# Autodesk Inventor assembly: Hebel_Klemme
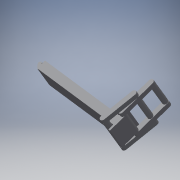
[picture p0: Inventor's stored thumbnail of the model, 180x180]
Saved by Autodesk Inventor 2018 (Build 220112000, 112)
## iProperties
Created: 2018-02-02
Part Number: Hebel_Klemme
Material: Generisch
Document SubType Name: Assembly
Designer: Julian
Author: Julian
## Documents named in this file (10)
- C:\Users\Julian\Desktop\Schule\5AHME\Diplomarbeit\Git\fuettr_prototype\Mechanical\Inventorskizzen\Hebel_Klemme.iam
- C:\Users\Julian\Desktop\Schule\5AHME\Diplomarbeit\Git\fuettr_prototype\Mechanical\Inventorskizzen\Hebel_KLemme_Hebel.ipt
- C:\Users\Julian\Desktop\Schule\5AHME\Diplomarbeit\Git\fuettr_prototype\Mechanical\Inventorskizzen\Hebel_Klemme_oben.ipt
- C:\Users\Julian\Desktop\Schule\5AHME\Diplomarbeit\Git\fuettr_prototype\Mechanical\Inventorskizzen\Hebel_Klemme_Rohrende.ipt
- C:\Users\Julian\Desktop\Schule\5AHME\Diplomarbeit\Git\fuettr_prototype\Mechanical\Inventorskizzen\Hebel_Klemme_unten.ipt
- C:\Users\Julian\Desktop\Schule\5AHME\Diplomarbeit\Git\fuettr_prototype\Mechanical\Inventorskizzen\Hebel_Röhre.ipt
- C:\Users\Julian\Desktop\Schule\5AHME\Diplomarbeit\Git\fuettr_prototype\Mechanical\Inventorskizzen\Klemme_Hebel_Entstück.ipt
- C:\Users\Julian\Desktop\Schule\5AHME\Diplomarbeit\Git\fuettr_prototype\Mechanical\Inventorskizzen\Stift_28mm.ipt
- C:\Users\Julian\Desktop\Schule\5AHME\Diplomarbeit\Git\fuettr_prototype\Mechanical\Inventorskizzen\Stift_20mm.ipt
- C:\Users\Julian\Desktop\Schule\5AHME\Diplomarbeit\Git\fuettr_prototype\Mechanical\Inventorskizzen\Stift_36mm.ipt
## Components (14 placed, 9 different names)
1. Hebel_KLemme_Hebel:1 — Drehbar:2, Starr:1, Drehbar:4, Drehbar:6, Drehbar:1, Starr:4, Starr:6
2. Hebel_KLemme_Hebel:2 — Drehbar:3, Drehbar:5
3. Hebel_Klemme_oben:1
4. Hebel_Klemme_Rohrende:1 — Starr:2, Starr:3
5. Hebel_Klemme_unten:1 — Drehbar:1, Drehbar:2, Drehbar:3, Starr:5
6. Hebel_Röhre:1 — Starr:1
7. Klemme_Hebel_Entstück:1 — Drehbar:5, Starr:2
8. Klemme_Hebel_Entstück:2 — Drehbar:4, Starr:3, Starr:7, Starr:8
9. Hebel_Röhre:2 — Drehbar:6
10. Stift_28mm:1 — Starr:4
11. Stift_20mm:1 — Starr:5
12. Stift_28mm:2 — Starr:6
13. Stift_36mm:1 — Starr:7
14. Stift_36mm:2 — Starr:8
## Relationships (14: WeldJoint 8, RevoluteJoint 6)
- Drehbar:1 [RevoluteJoint]: Hebel_KLemme_Hebel:1 ↔ Hebel_Klemme_unten:1
- Drehbar:2 [RevoluteJoint]: Hebel_KLemme_Hebel:1 ↔ Hebel_Klemme_unten:1
- Drehbar:3 [RevoluteJoint]: Hebel_KLemme_Hebel:2 ↔ Hebel_Klemme_unten:1
- Starr:1 [WeldJoint]: Hebel_KLemme_Hebel:1 ↔ Hebel_Röhre:1
- Drehbar:4 [RevoluteJoint]: Hebel_KLemme_Hebel:1 ↔ Klemme_Hebel_Entstück:2
- Drehbar:5 [RevoluteJoint]: Hebel_KLemme_Hebel:2 ↔ Klemme_Hebel_Entstück:1
- Starr:2 [WeldJoint]: Hebel_Klemme_Rohrende:1 ↔ Klemme_Hebel_Entstück:1
- Starr:3 [WeldJoint]: Hebel_Klemme_Rohrende:1 ↔ Klemme_Hebel_Entstück:2
- Drehbar:6 [RevoluteJoint]: Hebel_KLemme_Hebel:1 ↔ Hebel_Röhre:2
- Starr:4 [WeldJoint]: Hebel_KLemme_Hebel:1 ↔ Stift_28mm:1
- Starr:5 [WeldJoint]: Hebel_Klemme_unten:1 ↔ Stift_20mm:1
- Starr:6 [WeldJoint]: Hebel_KLemme_Hebel:1 ↔ Stift_28mm:2
- Starr:7 [WeldJoint]: Klemme_Hebel_Entstück:2 ↔ Stift_36mm:1
- Starr:8 [WeldJoint]: Klemme_Hebel_Entstück:2 ↔ Stift_36mm:2
